# Autodesk Inventor assembly: Cover-Frame-Assembly
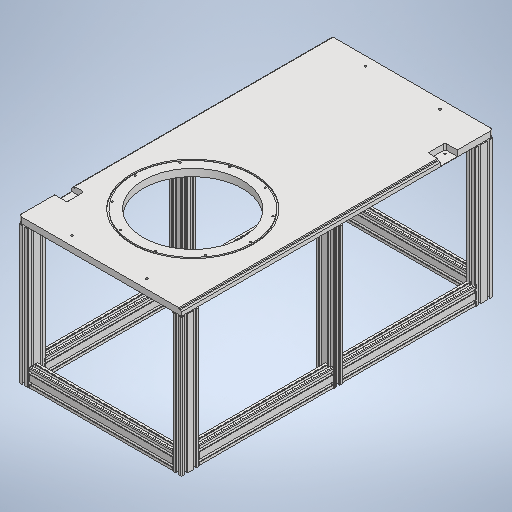
[picture p0: Inventor's stored thumbnail of the model, 512x512]
Saved by Autodesk Inventor 2025 (Build 290162000, 162)
## iProperties
Created: 2024-06-18
Part Number: Cover-Frame-Assembly
Document SubType Name: Assembly
Designer: mumin
Author: mumin
## Documents named in this file (5)
- C:\GitHub\In-situ-monitoring-of-powder-bed-fusion-additive-manufacturing\system_development\Orichalcum\v0.2\Hardware_design\custom-cover\Cover-Frame-Assembly.iam
- C:\GitHub\In-situ-monitoring-of-powder-bed-fusion-additive-manufacturing\system_development\Orichalcum\v0.2\Hardware_design\custom-cover\cover\Updated Cover.ipt
- C:\GitHub\In-situ-monitoring-of-powder-bed-fusion-additive-manufacturing\system_development\Orichalcum\v0.2\Hardware_design\custom-cover\8020-parts\20-40.ipt
- C:\GitHub\In-situ-monitoring-of-powder-bed-fusion-additive-manufacturing\system_development\Orichalcum\v0.2\Hardware_design\custom-cover\8020-parts\20-40_11.7.ipt
- C:\GitHub\In-situ-monitoring-of-powder-bed-fusion-additive-manufacturing\system_development\Orichalcum\v0.2\Hardware_design\custom-cover\8020-parts\20-40_12.5.ipt
## Components (13 placed, 4 different names)
1. Updated Cover:1 — Mate:1, Flush:1, Flush:2, Flush:3, Mate:2, Flush:4, Mate:3, Flush:5, Flush:6, Mate:4, Flush:7, Flush:8, Mate:5, Flush:9, Mate:6, Flush:10
2. 20-40:1 — Mate:1, Flush:1, Flush:2, Mate:11, Flush:13, Mate:13, Flush:19, Flush:20
3. 20-40:2 — Mate:3, Flush:5, Flush:6
4. 20-40:3 — Mate:4, Flush:7, Flush:8, Flush:12
5. 20-40:4 — Flush:3, Mate:2, Flush:4, Mate:12, Flush:11, Mate:14, Flush:21, Flush:22
6. 20-40:5 — Mate:5, Flush:9, Mate:9, Mate:10, Flush:14, Flush:15, Flush:16
7. 20-40:6 — Mate:6, Flush:10, Mate:7, Mate:8, Flush:17, Flush:18
8. 20-40_11.7:1 — Mate:8, Flush:12, Flush:18
9. 20-40_11.7:2 — Mate:7, Mate:12, Flush:11, Flush:17
10. 20-40_11.7:3 — Mate:9, Flush:14, Flush:15
11. 20-40_11.7:4 — Mate:10, Mate:11, Flush:13, Flush:16
12. 20-40_12.5:1 — Mate:13, Flush:19, Flush:20
13. 20-40_12.5:2 — Mate:14, Flush:21, Flush:22
## Relationships (36: Flush 22, Mate 14)
- Mate:1: Updated Cover:1 ↔ 20-40:1
- Flush:1: Updated Cover:1 ↔ 20-40:1
- Flush:2: Updated Cover:1 ↔ 20-40:1
- Flush:3: Updated Cover:1 ↔ 20-40:4
- Mate:2: Updated Cover:1 ↔ 20-40:4
- Flush:4: Updated Cover:1 ↔ 20-40:4
- Mate:3: Updated Cover:1 ↔ 20-40:2
- Flush:5: Updated Cover:1 ↔ 20-40:2
- Flush:6: Updated Cover:1 ↔ 20-40:2
- Mate:4: Updated Cover:1 ↔ 20-40:3
- Flush:7: Updated Cover:1 ↔ 20-40:3
- Flush:8: Updated Cover:1 ↔ 20-40:3
- Mate:5: Updated Cover:1 ↔ 20-40:5
- Flush:9: Updated Cover:1 ↔ 20-40:5
- Mate:6: Updated Cover:1 ↔ 20-40:6
- Flush:10: Updated Cover:1 ↔ 20-40:6
- Mate:7: 20-40:6 ↔ 20-40_11.7:2
- Mate:8: 20-40:6 ↔ 20-40_11.7:1
- Mate:9: 20-40:5 ↔ 20-40_11.7:3
- Mate:10: 20-40:5 ↔ 20-40_11.7:4
- Mate:11: 20-40:1 ↔ 20-40_11.7:4
- Mate:12: 20-40:4 ↔ 20-40_11.7:2
- Flush:11: 20-40:4 ↔ 20-40_11.7:2
- Flush:12: 20-40:3 ↔ 20-40_11.7:1
- Flush:13: 20-40:1 ↔ 20-40_11.7:4
- Flush:14: 20-40:5 ↔ 20-40_11.7:3
- Flush:15: 20-40:5 ↔ 20-40_11.7:3
- Flush:16: 20-40:5 ↔ 20-40_11.7:4
- Flush:17: 20-40:6 ↔ 20-40_11.7:2
- Flush:18: 20-40:6 ↔ 20-40_11.7:1
- Mate:13: 20-40:1 ↔ 20-40_12.5:1
- Flush:19: 20-40:1 ↔ 20-40_12.5:1
- Flush:20: 20-40:1 ↔ 20-40_12.5:1
- Mate:14: 20-40:4 ↔ 20-40_12.5:2
- Flush:21: 20-40:4 ↔ 20-40_12.5:2
- Flush:22: 20-40:4 ↔ 20-40_12.5:2
